# Autodesk Inventor assembly: DriveTrainSamdwich
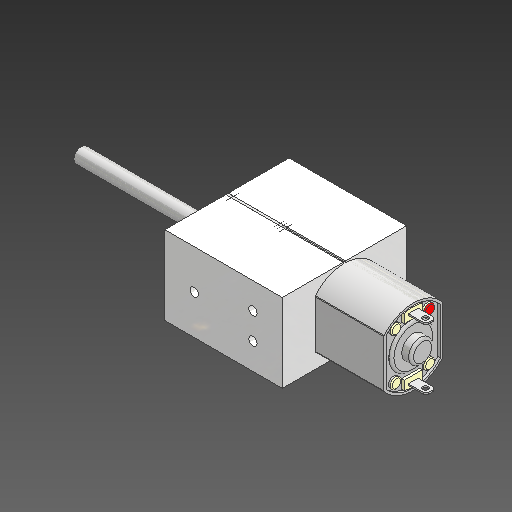
[picture p0: Inventor's stored thumbnail of the model, 512x512]
Saved by Autodesk Inventor 2021 (Build 250183000, 183)
## iProperties
Created: 2021-02-22
Part Number: DriveTrainSamdwich
Document SubType Name: Assembly
Designer: Esketitttttt
Mass: 30.8925 g
Surface Area: 73.4722 cm^2
Volume: 10.3836 cm^3
Density: 2.97514 g/cm^3
Author: Esketitttttt
## Documents named in this file (3)
- C:\Users\Esketitttttt\Documents\GrabCAD\Insomnia 2020\Versions\2 UHMW Mode\DriveTrainSamdwich.iam
- C:\Users\Esketitttttt\Documents\GrabCAD\Insomnia 2020\Versions\2 UHMW Mode\TopMotorMountSandwich3DPrint.ipt
- C:\Users\Esketitttttt\Documents\GrabCAD\Insomnia 2020\Versions\2 UHMW Mode\FingerTech_Silver_Spark_223350.ipt
## Components (3 placed, 2 different names)
1. TopMotorMountSandwich3DPrint:1 — Insert:1, Transitional:1
2. TopMotorMountSandwich3DPrint:2 — Insert:2, Transitional:2
3. FingerTech_Silver_Spark_223350:1 — Insert:1, Transitional:1, Insert:2, Transitional:2
## Relationships (4: Insert 2, Transitional 2)
- Insert:1: TopMotorMountSandwich3DPrint:1 ↔ FingerTech_Silver_Spark_223350:1
- Transitional:1: TopMotorMountSandwich3DPrint:1 ↔ FingerTech_Silver_Spark_223350:1
- Insert:2: TopMotorMountSandwich3DPrint:2 ↔ FingerTech_Silver_Spark_223350:1
- Transitional:2: TopMotorMountSandwich3DPrint:2 ↔ FingerTech_Silver_Spark_223350:1
